# Autodesk Inventor assembly: delta_1
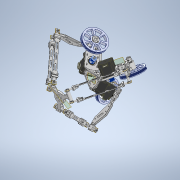
[picture p0: Inventor's stored thumbnail of the model, 180x180]
Saved by Autodesk Inventor 2020 (Build 240168000, 168)
## iProperties
Created: 2020-01-18
Part Number: delta_1
Document SubType Name: Assembly
Designer: psrobotics
Author: psrobotics
## Documents named in this file (13)
- F:\projects-3\delta arm\hardware\delta_1.iam
- F:\projects-3\delta arm\hardware\arm_shift_1.iam
- F:\projects-3\delta arm\hardware\arm_holder_1.ipt
- F:\projects-3\delta arm\hardware\arm_holder_2.ipt
- F:\projects-3\delta arm\hardware\arm_holder_3.ipt
- F:\projects-3\delta arm\hardware\arm_1.ipt
- F:\projects-3\delta arm\hardware\arm_2.ipt
- F:\projects-3\delta arm\hardware\arm_3.ipt
- F:\projects-3\delta arm\hardware\eye_bearing.iam
- F:\projects-3\delta arm\hardware\arm_5.ipt
- F:\projects-3\delta arm\hardware\end_holder.ipt
- F:\projects-3\delta arm\hardware\source\omron-ss-5gl-limit-switch-1.snapshot.1\OMRON_SS_5GL\OMRON_ss-5gl.iam
- F:\projects-3\delta arm\hardware\switch_holder.ipt
## Components (41 placed, 12 different names)
1. arm_shift_1:1 [sub-assembly] — Angle:1, Mate:2, Flush:3, Flush:6, Insert:2, Angle:4, Insert:5
2. arm_shift_1:2 [sub-assembly] — Angle:1, Angle:2, Mate:1, Flush:4, Flush:7, Insert:3, Angle:5, Insert:6, Mate:4, Angle:7, Tangent:1, Flush:17
3. arm_shift_1:3 [sub-assembly] — Angle:2, Mate:3, Flush:2, Flush:5, Flush:8, Insert:1, Angle:3, Insert:4
4. arm_holder_1:1 — Mate:1, Mate:2, Mate:3, Flush:2, Flush:3, Flush:4, Flush:5, Flush:6, Flush:7
5. arm_holder_2:1 — Flush:8, Insert:1, Angle:3, Flush:11
6. arm_holder_2:2 — Insert:2, Angle:4, Flush:9
7. arm_holder_2:3 — Insert:3, Angle:5, Flush:10
8. arm_holder_3:1 — Flush:9, Flush:10, Flush:11
9. arm_1:1 — Insert:4, Flush:12, Insert:7, Insert:8, Insert:12
10. arm_1:2 — Insert:5, Insert:22, Insert:23, Insert:24
11. arm_1:3 — Insert:6, Insert:16, Insert:17, Insert:18, Insert:61
12. arm_2:1 — Flush:12, Insert:7, Insert:8, Flush:13, Insert:9, Insert:10
13. arm_3:1 — Flush:13, Insert:9, Insert:10, Insert:11, Insert:25, Insert:26
14. arm_2:2 — Insert:11, Insert:12
15. arm_2:3 — Insert:16, Insert:17
16. arm_3:2 — Insert:45, Insert:47, Insert:62, Insert:63
17. arm_2:4 — Insert:18, Insert:61, Insert:62, Insert:63
18. arm_2:5 — Insert:22, Insert:23
19. arm_3:3 — Insert:57, Insert:59
20. arm_2:6 — Insert:24
21. eye_bearing:1 [sub-assembly] — Insert:25, Flush:16, Insert:27, Insert:28
22. eye_bearing:2 [sub-assembly] — Insert:26, Insert:33, Insert:34
23. arm_5:1 — Flush:16, Insert:27, Insert:28, Insert:29, Insert:30
24. eye_bearing:3 [sub-assembly] — Insert:29, Insert:30, Insert:36
25. arm_5:2 — Insert:33, Insert:34
26. eye_bearing:4 [sub-assembly] — Insert:35
27. end_holder:1 — Insert:35, Insert:36, Insert:46, Insert:48, Insert:58, Insert:60
28. eye_bearing:5 [sub-assembly] — Insert:45
29. arm_5:3
30. eye_bearing:6 [sub-assembly] — Insert:46
31. eye_bearing:7 [sub-assembly] — Insert:47
32. arm_5:4
33. eye_bearing:8 [sub-assembly] — Insert:48
34. eye_bearing:9 [sub-assembly] — Insert:59
35. arm_5:5
36. eye_bearing:10 [sub-assembly] — Insert:60
37. eye_bearing:11 [sub-assembly] — Insert:57
38. arm_5:6
39. eye_bearing:12 [sub-assembly] — Insert:58
40. OMRON_ss-5gl:1 [sub-assembly] — Mate:4, Angle:7, Tangent:1
41. switch_holder:1 — Flush:17
## Relationships (87: Insert 60, Flush 16, Angle 6, Mate 4, Tangent 1)
- Angle:1 (120 deg): arm_shift_1:1 ↔ arm_shift_1:2
- Angle:2 (240 deg): arm_shift_1:2 ↔ arm_shift_1:3
- Flush:1
- Mate:1: arm_shift_1:2 ↔ arm_holder_1:1
- Mate:2: arm_shift_1:1 ↔ arm_holder_1:1
- Mate:3: arm_shift_1:3 ↔ arm_holder_1:1
- Flush:2: arm_shift_1:3 ↔ arm_holder_1:1
- Flush:3: arm_shift_1:1 ↔ arm_holder_1:1
- Flush:4: arm_shift_1:2 ↔ arm_holder_1:1
- Flush:5 (5 mm): arm_shift_1:3 ↔ arm_holder_1:1
- Flush:6 (5 mm): arm_shift_1:1 ↔ arm_holder_1:1
- Flush:7 (5 mm): arm_shift_1:2 ↔ arm_holder_1:1
- Flush:8: arm_shift_1:3 ↔ arm_holder_2:1
- Insert:1: arm_shift_1:3 ↔ arm_holder_2:1
- Angle:3 (0 deg): arm_shift_1:3 ↔ arm_holder_2:1
- Insert:2: arm_shift_1:1 ↔ arm_holder_2:2
- Angle:4 (0 deg): arm_shift_1:1 ↔ arm_holder_2:2
- Insert:3: arm_shift_1:2 ↔ arm_holder_2:3
- Angle:5 (0 deg): arm_shift_1:2 ↔ arm_holder_2:3
- Flush:9: arm_holder_2:2 ↔ arm_holder_3:1
- Flush:10: arm_holder_2:3 ↔ arm_holder_3:1
- Flush:11: arm_holder_2:1 ↔ arm_holder_3:1
- Insert:4 (3 mm): arm_shift_1:3 ↔ arm_1:1
- Insert:5 (3 mm): arm_shift_1:1 ↔ arm_1:2
- Insert:6 (3 mm): arm_shift_1:2 ↔ arm_1:3
- Flush:12: arm_1:1 ↔ arm_2:1
- Insert:7: arm_1:1 ↔ arm_2:1
- Insert:8: arm_1:1 ↔ arm_2:1
- Flush:13: arm_2:1 ↔ arm_3:1
- Insert:9: arm_2:1 ↔ arm_3:1
- Insert:10: arm_2:1 ↔ arm_3:1
- Insert:11: arm_3:1 ↔ arm_2:2
- Insert:12: arm_1:1 ↔ arm_2:2
- Insert:16: arm_1:3 ↔ arm_2:3
- Insert:17: arm_1:3 ↔ arm_2:3
- Insert:18: arm_1:3 ↔ arm_2:4
- [Flush]: arm_2:5 ↔ arm_3:3
- [Insert]: arm_2:5 ↔ arm_3:3
- [Insert]: arm_2:5 ↔ arm_3:3
- [Insert]: arm_3:3 ↔ arm_2:6
- Insert:22: arm_1:2 ↔ arm_2:5
- Insert:23: arm_1:2 ↔ arm_2:5
- Insert:24: arm_1:2 ↔ arm_2:6
- Insert:25: arm_3:1 ↔ eye_bearing:1
- Insert:26: arm_3:1 ↔ eye_bearing:2
- Flush:16: eye_bearing:1 ↔ arm_5:1
- Insert:27: eye_bearing:1 ↔ arm_5:1
- Insert:28: eye_bearing:1 ↔ arm_5:1
- Insert:29: arm_5:1 ↔ eye_bearing:3
- Insert:30: arm_5:1 ↔ eye_bearing:3
- [Insert]: arm_5:2 ↔ eye_bearing:4
- [Insert]: arm_5:2 ↔ eye_bearing:4
- Insert:33: eye_bearing:2 ↔ arm_5:2
- Insert:34: eye_bearing:2 ↔ arm_5:2
- Insert:35: eye_bearing:4 ↔ end_holder:1
- Insert:36: eye_bearing:3 ↔ end_holder:1
- [Insert]: arm_5:3 ↔ eye_bearing:6
- [Insert]: arm_5:3 ↔ eye_bearing:6
- [Insert]: eye_bearing:5 ↔ arm_5:3
- [Insert]: eye_bearing:5 ↔ arm_5:3
- [Insert]: arm_5:4 ↔ eye_bearing:8
- [Insert]: arm_5:4 ↔ eye_bearing:8
- [Insert]: eye_bearing:7 ↔ arm_5:4
- [Insert]: eye_bearing:7 ↔ arm_5:4
- Insert:45: arm_3:2 ↔ eye_bearing:5
- Insert:46: end_holder:1 ↔ eye_bearing:6
- Insert:47: arm_3:2 ↔ eye_bearing:7
- Insert:48: end_holder:1 ↔ eye_bearing:8
- [Insert]: arm_5:5 ↔ eye_bearing:10
- [Insert]: arm_5:5 ↔ eye_bearing:10
- [Insert]: eye_bearing:9 ↔ arm_5:5
- [Insert]: eye_bearing:9 ↔ arm_5:5
- [Insert]: arm_5:6 ↔ eye_bearing:12
- [Insert]: arm_5:6 ↔ eye_bearing:12
- [Insert]: eye_bearing:11 ↔ arm_5:6
- [Insert]: eye_bearing:11 ↔ arm_5:6
- Insert:57: arm_3:3 ↔ eye_bearing:11
- Insert:58: end_holder:1 ↔ eye_bearing:12
- Insert:59: arm_3:3 ↔ eye_bearing:9
- Insert:60: end_holder:1 ↔ eye_bearing:10
- Insert:61: arm_1:3 ↔ arm_2:4
- Mate:4 (5 mm): arm_shift_1:2 ↔ OMRON_ss-5gl:1
- Angle:7 (135 deg): arm_shift_1:2 ↔ OMRON_ss-5gl:1
- Tangent:1 (-0.25 mm): arm_shift_1:2 ↔ OMRON_ss-5gl:1
- Flush:17: arm_shift_1:2 ↔ switch_holder:1
- Insert:62: arm_3:2 ↔ arm_2:4
- Insert:63: arm_3:2 ↔ arm_2:4
## Named parameters: d43_d31 = 0 mm, d44_d32 = 0 mm, d45_d33 = 0 mm, d46_d34 = 0 mm, d57_d55 = 0 mm, d58_d56 = 0 mm, d63_d57_d55 = 0 mm, d64_d58_d56 = 0 mm, d65_d59 = 0 mm, d66_d60 = 0 mm, d67_d57_d55 = 0 mm, d68_d58_d56 = 0 mm, d69_d59 = 0 mm, d70_d60 = 0 mm, d75_d57_d55 = 0 mm, d76_d58_d56 = 0 mm, d77_d59 = 0 mm, d78_d60 = 0 mm, d79_d57_d55 = 0 mm, d80_d58_d56 = 0 mm, d81_d59 = 0 mm, d82_d60 = 0 mm
